# Autodesk Inventor assembly: Assembly1
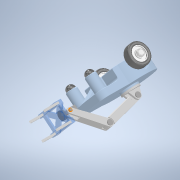
[picture p0: Inventor's stored thumbnail of the model, 180x180]
Saved by Autodesk Inventor 2021 (Build 250183000, 183)
## iProperties
Created: 2021-08-03
Part Number: Assembly1
Document SubType Name: Assembly
Designer: hp
Author: hp
## Documents named in this file (15)
- C:\Users\hp\Desktop\Assembly2.iam
- C:\Users\hp\Desktop\New_version\New_Body_Frame.ipt
- C:\Users\hp\Desktop\New_version\New_Main_Axle.ipt
- C:\Users\hp\Desktop\New_version\New_main_wheel.ipt
- C:\Users\hp\Desktop\New_version\New_Tire.ipt
- C:\Users\hp\Desktop\Final_version\New_Arm_plate.ipt
- C:\Users\hp\Desktop\Final_version\New_ThinArm_first.ipt
- C:\Users\hp\Desktop\Final_version\New_ThinArm_second.ipt
- C:\Users\hp\Desktop\Final_version\New_ThinAxle1.ipt
- C:\Users\hp\Desktop\Final_version\New_ThinAxle2.ipt
- C:\Users\hp\Desktop\Final_version\New_ThinFinger.ipt
- C:\Users\hp\Desktop\Final_version\New_ThinGripper_base.ipt
- C:\Users\hp\Desktop\Final_version\New_ThinGripper.ipt
- C:\Users\hp\Desktop\Final_version\gasket.ipt
- C:\Users\hp\Desktop\Final_version\Universal_Wheel.ipt
## Components (23 placed, 14 different names)
1. New_Body_Frame:1 — Mate:1, Mate:2, Mate:9, Mate:10, Mate:41, Mate:42, Mate:43, Mate:44
2. New_Main_Axle:1 — Mate:1, Mate:2, Mate:3, Mate:4, Mate:5, Mate:6, Mate:7, Mate:8
3. New_main_wheel:1 — Mate:3, Mate:5, Flush:2
4. New_main_wheel:2 — Mate:4, Mate:6, Flush:1
5. New_Tire:1 — Mate:8, Flush:2
6. New_Tire:2 — Mate:7, Flush:1
7. New_Arm_plate:1 — Mate:9, Mate:10, Mate:13, Mate:14, Mate:17
8. New_ThinAxle1:1 — Mate:13, Mate:14, Mate:16
9. New_ThinAxle2:1 — Mate:19, Mate:20
10. New_ThinFinger:1 — Mate:33, Mate:34
11. New_ThinFinger:2 — Mate:35, Mate:36
12. New_ThinFinger:3 — Mate:39, Mate:40
13. New_ThinFinger:4 — Mate:37, Mate:38
14. New_ThinGripper_base:1 — Mate:21, Mate:30, Mate:31, Mate:32
15. New_ThinGripper:1 — Mate:31, Mate:32, Mate:33, Mate:34, Mate:35, Mate:36, Mate:37, Mate:38, Mate:39, Mate:40
16. New_ThinArm_first:1 — Mate:15, Mate:16, Mate:17, Mate:18
17. New_ThinArm_second:1 — Mate:15, Mate:18, Mate:19, Mate:20, Mate:21, Mate:22, Mate:23, Mate:24, Mate:25, Mate:26, Mate:27, Mate:28, Mate:29
18. gasket:1 — Mate:22, Mate:28, Mate:30
19. gasket:2 — Mate:23, Mate:29
20. gasket:3 — Mate:24, Mate:27
21. gasket:4 — Mate:25, Mate:26
22. Universal_Wheel:1 — Mate:43, Mate:44
23. Universal_Wheel:2 — Mate:41, Mate:42
## Relationships (44: Mate 42, Flush 2)
- Mate:1: New_Body_Frame:1 ↔ New_Main_Axle:1
- Mate:2 (5.2 mm): New_Body_Frame:1 ↔ New_Main_Axle:1
- Mate:3: New_Main_Axle:1 ↔ New_main_wheel:1
- Mate:4: New_Main_Axle:1 ↔ New_main_wheel:2
- Mate:5: New_Main_Axle:1 ↔ New_main_wheel:1
- Mate:6: New_Main_Axle:1 ↔ New_main_wheel:2
- Mate:7: New_Main_Axle:1 ↔ New_Tire:2
- Mate:8: New_Main_Axle:1 ↔ New_Tire:1
- Flush:1 (-0.2 mm): New_main_wheel:2 ↔ New_Tire:2
- Flush:2 (-0.2 mm): New_main_wheel:1 ↔ New_Tire:1
- Mate:9: New_Body_Frame:1 ↔ New_Arm_plate:1
- Mate:10: New_Body_Frame:1 ↔ New_Arm_plate:1
- Mate:13: New_Arm_plate:1 ↔ New_ThinAxle1:1
- Mate:14: New_Arm_plate:1 ↔ New_ThinAxle1:1
- Mate:15: New_ThinArm_first:1 ↔ New_ThinArm_second:1
- Mate:16: New_ThinAxle1:1 ↔ New_ThinArm_first:1
- Mate:17: New_Arm_plate:1 ↔ New_ThinArm_first:1
- Mate:18: New_ThinArm_first:1 ↔ New_ThinArm_second:1
- Mate:19: New_ThinAxle2:1 ↔ New_ThinArm_second:1
- Mate:20: New_ThinAxle2:1 ↔ New_ThinArm_second:1
- Mate:21: New_ThinGripper_base:1 ↔ New_ThinArm_second:1
- Mate:22: New_ThinArm_second:1 ↔ gasket:1
- Mate:23: New_ThinArm_second:1 ↔ gasket:2
- Mate:24: New_ThinArm_second:1 ↔ gasket:3
- Mate:25: New_ThinArm_second:1 ↔ gasket:4
- Mate:26: New_ThinArm_second:1 ↔ gasket:4
- Mate:27: New_ThinArm_second:1 ↔ gasket:3
- Mate:28: New_ThinArm_second:1 ↔ gasket:1
- Mate:29: New_ThinArm_second:1 ↔ gasket:2
- Mate:30: New_ThinGripper_base:1 ↔ gasket:1
- Mate:31: New_ThinGripper_base:1 ↔ New_ThinGripper:1
- Mate:32: New_ThinGripper_base:1 ↔ New_ThinGripper:1
- Mate:33: New_ThinFinger:1 ↔ New_ThinGripper:1
- Mate:34: New_ThinFinger:1 ↔ New_ThinGripper:1
- Mate:35: New_ThinFinger:2 ↔ New_ThinGripper:1
- Mate:36: New_ThinFinger:2 ↔ New_ThinGripper:1
- Mate:37: New_ThinFinger:4 ↔ New_ThinGripper:1
- Mate:38: New_ThinFinger:4 ↔ New_ThinGripper:1
- Mate:39: New_ThinFinger:3 ↔ New_ThinGripper:1
- Mate:40: New_ThinFinger:3 ↔ New_ThinGripper:1
- Mate:41: New_Body_Frame:1 ↔ Universal_Wheel:2
- Mate:42: New_Body_Frame:1 ↔ Universal_Wheel:2
- Mate:43: New_Body_Frame:1 ↔ Universal_Wheel:1
- Mate:44: New_Body_Frame:1 ↔ Universal_Wheel:1
